# Autodesk Inventor assembly: 双四方头洞
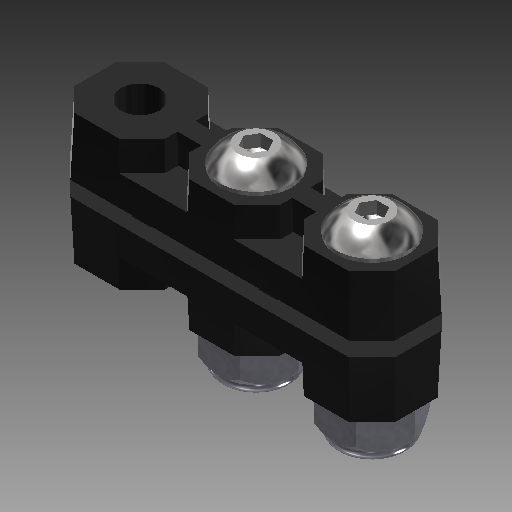
[picture p0: Inventor's stored thumbnail of the model, 512x512]
Saved by Autodesk Inventor 2019.3 (Build 233278000, 278)
## iProperties
Created: 2018-09-09
Part Number: 双四方头洞
Material: 常规
Document SubType Name: Assembly
Designer: aresp
Mass: 11.6155 g
Surface Area: 44.4845 cm^2
Volume: 4.06855 cm^3
Density: 2.85495 g/cm^3
Author: aresp
## Documents named in this file (4)
- D:\cad\工作空间\双四方头洞.iam
- D:\cad\零件库\Bearing Flat.ipt
- D:\cad\零件库\螺丝螺帽\Screw 8-32 x 0.750'' - Black.ipt
- D:\cad\零件库\螺丝螺帽\Nut 8-32 Nylock.ipt
## Components (6 placed, 3 different names)
1. Bearing Flat:1
2. Bearing Flat:2
3. Screw 8-32 x 0.750'' - Black:1
4. Screw 8-32 x 0.750'' - Black:2
5. Nut 8-32 Nylock:1
6. Nut 8-32 Nylock:2
## Relationships (5: Insert 4, Mate 1)
- [Mate]: Bearing Flat:1 ↔ Bearing Flat:2
- [Insert]: Bearing Flat:1 ↔ Screw 8-32 x 0.750'' - Black:1
- [Insert]: Bearing Flat:1 ↔ Screw 8-32 x 0.750'' - Black:2
- [Insert]: Bearing Flat:2 ↔ Nut 8-32 Nylock:1
- [Insert]: Bearing Flat:2 ↔ Nut 8-32 Nylock:2
